# Autodesk Inventor assembly: VSR20A-T3
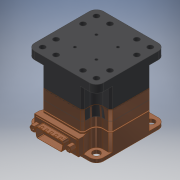
[picture p0: Inventor's stored thumbnail of the model, 180x180]
Saved by Autodesk Inventor 2018.2 (Build 222227000, 227)
## iProperties
Created: 2014-12-02
Vendor: ZABER
Document SubType Name: Assembly
Designer: ARNOLDJ
Mass: 261.327 g
Surface Area: 412.56 cm^2
Volume: 261.327 cm^3
Density: 1 g/cm^3
Part Number: VSR20A-T3
Description: MOTORIZED LIFT STAGE, 20MM TRAVEL, FINE RESOLUTION
RuleStatus: InUse
AfterDocSave0: file://Part Number Cleaner
DESIGN DEPARTMENT: HHMI: JFRC - ID&F
ALTERED ITEM PART NUMBER: N/A
ALTERED ITEM VENDOR: N/A
ALTERED ITEM DESCRIPTION: N/A
Revision Number: 0
## Documents named in this file (3)
- C:\_WORKSPACE\DATA\PROJECTS\_PROJECTS BY LAB\SVOBODA (LAB)\MOUSE POSITIONING SYSTEMS\MCAD\BALL SETUP\VSR-T3.iam
- C:\_WORKSPACE\DATA\PROJECTS\_PROJECTS BY LAB\SVOBODA (LAB)\MOUSE POSITIONING SYSTEMS\MCAD\BALL SETUP\VSR-T3.ipt
- C:\_WORKSPACE\DATA\PROJECTS\_PROJECTS BY LAB\SVOBODA (LAB)\MOUSE POSITIONING SYSTEMS\MCAD\BALL SETUP\VSR-T3 Upper.ipt
## Components (2 placed, 2 different names)
1. VSR-T3:1 — Flush:3, Flush:4, Mate:1, Angle:1
2. VSR-T3 Upper:1 — Flush:1, Flush:2, Flush:3, Flush:4, Mate:1, Angle:1
## Relationships (6: Flush 4, Mate 1, Angle 1)
- Flush:1: VSR-T3 Upper:1
- Flush:2: VSR-T3 Upper:1
- Flush:3 (10 mm): VSR-T3:1 ↔ VSR-T3 Upper:1
- Flush:4: VSR-T3:1 ↔ VSR-T3 Upper:1
- Mate:1: VSR-T3:1 ↔ VSR-T3 Upper:1
- Angle:1 (0 deg): VSR-T3:1 ↔ VSR-T3 Upper:1
